# Autodesk Inventor assembly: viaductpillertest
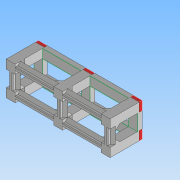
[picture p0: Inventor's stored thumbnail of the model, 180x180]
Saved by Autodesk Inventor 2021 (Build 250183000, 183)
## iProperties
Created: 2021-03-15
Part Number: viaductpillertest
Document SubType Name: Assembly
Designer: kumagai
Author: kumagai
## Documents named in this file (2)
- Z:\Develop\CAD\PlaRails\Slope\viaductpillertest.iam
- Z:\Develop\CAD\PlaRails\Slope\ViaductPillarsUnit.ipt
## Components (2 placed, 1 different names)
1. ViaductPillarsUnit:1 — フラッシュ:1, フラッシュ:2
2. ViaductPillarsUnit:2 — フラッシュ:1, フラッシュ:2
## Relationships (2: Flush 2)
- フラッシュ:1 [Flush]: ViaductPillarsUnit:1 ↔ ViaductPillarsUnit:2
- フラッシュ:2 [Flush]: ViaductPillarsUnit:1 ↔ ViaductPillarsUnit:2
